# Autodesk Inventor assembly: plateau moteurs
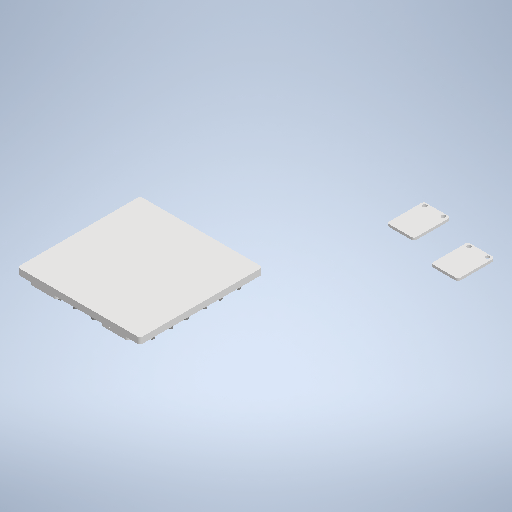
[picture p0: Inventor's stored thumbnail of the model, 512x512]
Saved by Autodesk Inventor 2025.2 (Build 292293000, 293)
## iProperties
Created: 2025-02-17
Part Number: plateau moteurs
Document SubType Name: Assembly
Designer: antoi
Author: antoi
## Documents named in this file (3)
- C:\Users\antoi\Documents\Henallux_24_25\Q2\proj\prototype\plateau moteurs.iam
- C:\Users\antoi\Documents\Henallux_24_25\Q2\proj\prototype\DFR0440.ipt
- C:\Users\antoi\Documents\Henallux_24_25\Q2\proj\prototype\plateau.ipt
## Components (5 placed, 2 different names)
1. DFR0440:1 — Placage:1, Affleurement:1, Affleurement:2
2. DFR0440:2 — Placage:2, Affleurement:3, Affleurement:4
3. DFR0440:3
4. DFR0440:4
5. plateau:1 — Placage:1, Placage:2, Affleurement:1, Affleurement:2, Affleurement:3, Affleurement:4
## Relationships (6: Flush 4, Mate 2)
- Placage:1 [Mate]: DFR0440:1 ↔ plateau:1
- Placage:2 [Mate]: DFR0440:2 ↔ plateau:1
- Affleurement:1 [Flush] (10 mm): DFR0440:1 ↔ plateau:1
- Affleurement:2 [Flush]: DFR0440:1 ↔ plateau:1
- Affleurement:3 [Flush]: DFR0440:2 ↔ plateau:1
- Affleurement:4 [Flush] (10 mm): DFR0440:2 ↔ plateau:1
